# Autodesk Inventor assembly: 組合2
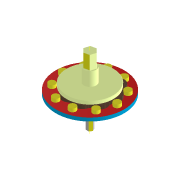
[picture p0: Inventor's stored thumbnail of the model, 180x180]
Saved by Autodesk Inventor 2022 (Build 260153000, 153)
## iProperties
Created: 2023-05-23
Part Number: 組合2
Document SubType Name: Assembly
Designer: JOU
Author: JOU
## Documents named in this file (5)
- C:\Users\JOU\Desktop\git\Special-project\接觸解析器練習資料夾\接觸解析器練習資料夾\Cycloidal Gear\組合2.iam
- C:\Users\JOU\Desktop\git\Special-project\接觸解析器練習資料夾\接觸解析器練習資料夾\Cycloidal Gear\180219-Base.ipt
- C:\Users\JOU\Desktop\git\Special-project\接觸解析器練習資料夾\接觸解析器練習資料夾\Cycloidal Gear\180219-Disk.ipt
- C:\Users\JOU\Desktop\git\Special-project\接觸解析器練習資料夾\接觸解析器練習資料夾\Cycloidal Gear\180219-InputShaft.ipt
- C:\Users\JOU\Desktop\git\Special-project\接觸解析器練習資料夾\接觸解析器練習資料夾\Cycloidal Gear\180219-OutputShaft.ipt
## Components (4 placed, 4 different names)
1. 180219-Disk:1 — 貼合:3, 齊平:1, 貼合:4
2. 180219-InputShaft:1 — 貼合:1, 貼合:3, 齊平:1, 角度:1
3. 180219-OutputShaft:1 — 貼合:2, 貼合:5
4. 180219-Base:2 — 貼合:1, 貼合:2, 貼合:4, 貼合:5
## Relationships (7: Mate 5, Flush 1, Angle 1)
- 貼合:1 [Mate]: 180219-InputShaft:1 ↔ 180219-Base:2
- 貼合:2 [Mate]: 180219-OutputShaft:1 ↔ 180219-Base:2
- 貼合:3 [Mate]: 180219-Disk:1 ↔ 180219-InputShaft:1
- 齊平:1 [Flush]: 180219-Disk:1 ↔ 180219-InputShaft:1
- 貼合:4 [Mate]: 180219-Disk:1 ↔ 180219-Base:2
- 貼合:5 [Mate]: 180219-OutputShaft:1 ↔ 180219-Base:2
- 角度:1 [Angle] (0 deg): 180219-InputShaft:1
